# Autodesk Inventor assembly: Incubation_box
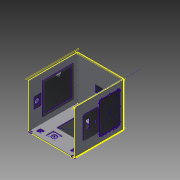
[picture p0: Inventor's stored thumbnail of the model, 180x180]
Saved by Autodesk Inventor 2015 SP2 (Build 190223200, 223)
## iProperties
Company: Newcastle University - Holden lab
Created: 2016-11-11
Part Number: Incubation_box
Document SubType Name: Assembly
Designer: Yann Cesbron
Mass: 18848.8 g
Surface Area: 42757.2 cm^2
Volume: 18848.8 cm^3
Density: 1 g/cm^3
Author: Yann Cesbron
## Documents named in this file (6)
- C:\temp\Users_shared\_PALM_scope_incubation_box_2_170409\Incubation_box.iam
- C:\temp\Users_shared\_PALM_scope_incubation_box_2_170409\Front_part.ipt
- C:\temp\Users_shared\_PALM_scope_incubation_box_2_170409\Right_side.ipt
- C:\temp\Users_shared\_PALM_scope_incubation_box_2_170409\Left_side.ipt
- C:\temp\Users_shared\_PALM_scope_incubation_box_2_170409\Back_part.ipt
- C:\temp\Users_shared\_PALM_scope_incubation_box_2_170409\Top_part.ipt
## Components (5 placed, 5 different names)
1. Front_panel:1 — Flush:1, Flush:2, Flush:3, Flush:4, Flush:8, Flush:10, Mate:1, Mate:2
2. Right_panel:1 — Flush:1, Flush:2, Flush:5, Flush:6, Flush:7, Mate:1
3. Left_panel:1 — Flush:3, Flush:4, Mate:2, Mate:3, Mate:4
4. Back_panel:1 — Flush:5, Flush:6, Flush:7, Mate:3
5. Top_panel:1 — Flush:8, Flush:10, Mate:4
## Relationships (13: Flush 9, Mate 4)
- Flush:1: Front_panel:1 ↔ Right_panel:1
- Flush:2: Front_panel:1 ↔ Right_panel:1
- Flush:3: Front_panel:1 ↔ Left_panel:1
- Flush:4: Front_panel:1 ↔ Left_panel:1
- Flush:5: Right_panel:1 ↔ Back_panel:1
- Flush:6: Right_panel:1 ↔ Back_panel:1
- Flush:7: Right_panel:1 ↔ Back_panel:1
- Flush:8: Front_panel:1 ↔ Top_panel:1
- Flush:10: Front_panel:1 ↔ Top_panel:1
- Mate:1: Front_panel:1 ↔ Right_panel:1
- Mate:2: Front_panel:1 ↔ Left_panel:1
- Mate:3: Left_panel:1 ↔ Back_panel:1
- Mate:4: Left_panel:1 ↔ Top_panel:1
